# Autodesk Inventor assembly: 总装配
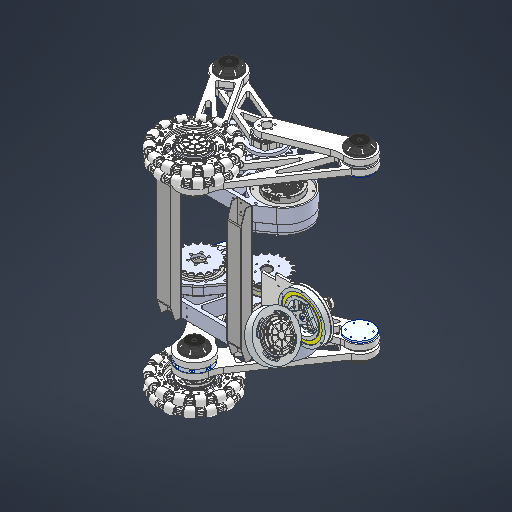
[picture p0: Inventor's stored thumbnail of the model, 512x512]
Saved by Autodesk Inventor 2025 (Build 290162000, 162)
## iProperties
Created: 2025-04-19
Part Number: 总装配
Document SubType Name: Assembly
Designer: XH
Author: XH
## Documents named in this file (4)
- C:\1A_Engineering_files\RCInventor\铝件版本\总装配.iam
- C:\1A_Engineering_files\RCInventor\铝件版本\装配体2_MIR1.iam
- C:\1A_Engineering_files\RCInventor\铝件版本\铝方管\40x15_MIR.ipt
- C:\1A_Engineering_files\RCInventor\铝件版本\轮系\舵轮\RMDL2.0——00.iam
## Components (5 placed, 3 different names)
1. 装配体2_MIR1:1 [sub-assembly] — 表面齐平:7, 表面齐平:8, 配合:10, 配合:14, 配合:15, 配合:16
2. 40x15_MIR:1 — 表面齐平:7, 表面齐平:8, 配合:10, 配合:11, 配合:12, 配合:13
3. 装配体2_MIR1:2 [sub-assembly] — 配合:11, 配合:12, 配合:13
4. 40x15_MIR:2 — 配合:14, 配合:15, 配合:16, 配合:17, 配合:18
5. RMDL2.0——00:1 [sub-assembly] — 配合:17, 配合:18
## Relationships (12: Mate 9, Flush 3)
- 表面齐平:1 [Flush] (138 mm)
- 表面齐平:7 [Flush]: 装配体2_MIR1:1 ↔ 40x15_MIR:1
- 表面齐平:8 [Flush]: 装配体2_MIR1:1 ↔ 40x15_MIR:1
- 配合:10 [Mate]: 装配体2_MIR1:1 ↔ 40x15_MIR:1
- 配合:11 [Mate]: 40x15_MIR:1 ↔ 装配体2_MIR1:2
- 配合:12 [Mate]: 40x15_MIR:1 ↔ 装配体2_MIR1:2
- 配合:13 [Mate]: 40x15_MIR:1 ↔ 装配体2_MIR1:2
- 配合:14 [Mate]: 装配体2_MIR1:1 ↔ 40x15_MIR:2
- 配合:15 [Mate]: 装配体2_MIR1:1 ↔ 40x15_MIR:2
- 配合:16 [Mate]: 装配体2_MIR1:1 ↔ 40x15_MIR:2
- 配合:17 [Mate]: 40x15_MIR:2 ↔ RMDL2.0——00:1
- 配合:18 [Mate] (50 mm): 40x15_MIR:2 ↔ RMDL2.0——00:1
